# Autodesk Inventor assembly: Structure
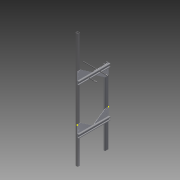
[picture p0: Inventor's stored thumbnail of the model, 180x180]
Saved by Autodesk Inventor 2015 SP1 (Build 190203100, 203)
## iProperties
Created: 2015-01-24
Part Number: Structure
Document SubType Name: Assembly
Designer: Peter
Author: Peter
## Documents named in this file (9)
- C:\Users\Brian\Documents\GitHub\FIRST-Team-1719-CAD-Team\2015 Robot CAD\Devices\Extender\Structure\Structure.iam
- C:\Users\Brian\Documents\GitHub\FIRST-Team-1719-CAD-Team\2015 Robot CAD\Lifter Super Structure\Tower\H-Shaped-Assembly\Horizontal-Unistrut-Tower-Connector-19-25.ipt
- C:\Users\Brian\Documents\GitHub\FIRST-Team-1719-CAD-Team\2015 Robot CAD\Devices\Extender\Structure\Horizontal-Unistrut-Tower-Connector-15.ipt
- C:\Users\Brian\Documents\GitHub\FIRST-Team-1719-CAD-Team\2015 Robot CAD\Devices\Extender\Structure\Square.ipt
- C:\Users\Brian\Documents\GitHub\FIRST-Team-1719-CAD-Team\2015 Robot CAD\Devices\Extender\Structure\Corner-Tower-Brace.ipt
- C:\Users\Brian\Documents\GitHub\FIRST-Team-1719-CAD-Team\2015 Robot CAD\Devices\Extender\Structure\Corner-Tower-Brace-Upper.ipt
- C:\Users\Brian\Documents\GitHub\FIRST-Team-1719-CAD-Team\2015 Robot CAD\Devices\Extender\Structure\3 8 Threaded Shaft.ipt
- C:\Users\Brian\Documents\GitHub\FIRST-Team-1719-CAD-Team\2015 Robot CAD\Devices\Extender\Structure\3 8 Threaded Shaft Pivot.ipt
- C:\Users\Brian\Documents\GitHub\FIRST-Team-1719-CAD-Team\2015 Robot CAD\Devices\Extender\Structure\3 8 Nut.ipt
## Components (18 placed, 8 different names)
1. Horizontal-Unistrut-Tower-Connector-19-25:1 — Flush:17, Mate:66, Mate:95
2. Horizontal-Unistrut-Tower-Connector-15:1 — Flush:17, Flush:18, Flush:19, Mate:73, Mate:90, Mate:92
3. Square:1 — Flush:24
4. Horizontal-Unistrut-Tower-Connector-15:2 — Flush:18, Flush:19, Mate:61, Mate:64
5. Corner-Tower-Brace:1 — Mate:61, Mate:66
6. Corner-Tower-Brace:4 — Mate:64
7. Corner-Tower-Brace-Upper:1 — Mate:73, Mate:76, Mate:86
8. Corner-Tower-Brace-Upper:2 — Mate:95, Mate:96, Mate:97
9. 3 8 Threaded Shaft:2 — Mate:76, Mate:84, Flush:25
10. 3 8 Threaded Shaft Pivot:1 — Mate:83, Flush:26, Mate:97
11. 3 8 Nut:1 — Mate:82, Mate:92
12. 3 8 Nut:2 — Mate:81, Mate:82, Mate:83, Mate:96
13. 3 8 Nut:3 — Mate:80, Flush:26
14. 3 8 Nut:4 — Mate:80, Mate:81
15. 3 8 Nut:5 — Mate:77, Mate:90
16. 3 8 Nut:6 — Mate:77, Mate:78
17. 3 8 Nut:7 — Mate:78, Mate:79, Mate:84, Mate:86
18. 3 8 Nut:8 — Mate:79, Flush:25
## Relationships (30: Mate 24, Flush 6)
- Mate:39
- Mate:40
- Mate:41
- Mate:42
- Mate:47
- Flush:17: Horizontal-Unistrut-Tower-Connector-19-25:1 ↔ Horizontal-Unistrut-Tower-Connector-15:1
- Flush:18: Horizontal-Unistrut-Tower-Connector-15:1 ↔ Horizontal-Unistrut-Tower-Connector-15:2
- Flush:19: Horizontal-Unistrut-Tower-Connector-15:1 ↔ Horizontal-Unistrut-Tower-Connector-15:2
- Mate:61: Horizontal-Unistrut-Tower-Connector-15:2 ↔ Corner-Tower-Brace:1
- Mate:64: Horizontal-Unistrut-Tower-Connector-15:2 ↔ Corner-Tower-Brace:4
- Mate:66: Horizontal-Unistrut-Tower-Connector-19-25:1 ↔ Corner-Tower-Brace:1
- Flush:24 (-12.7 mm): Square:1
- Mate:73: Horizontal-Unistrut-Tower-Connector-15:1 ↔ Corner-Tower-Brace-Upper:1
- Mate:76: Corner-Tower-Brace-Upper:1 ↔ 3 8 Threaded Shaft:2
- Mate:77: 3 8 Nut:5 ↔ 3 8 Nut:6
- Mate:78: 3 8 Nut:6 ↔ 3 8 Nut:7
- Mate:79: 3 8 Nut:7 ↔ 3 8 Nut:8
- Mate:80: 3 8 Nut:3 ↔ 3 8 Nut:4
- Mate:81: 3 8 Nut:2 ↔ 3 8 Nut:4
- Mate:82: 3 8 Nut:1 ↔ 3 8 Nut:2
- Mate:83: 3 8 Threaded Shaft Pivot:1 ↔ 3 8 Nut:2
- Mate:84: 3 8 Threaded Shaft:2 ↔ 3 8 Nut:7
- Mate:86: Corner-Tower-Brace-Upper:1 ↔ 3 8 Nut:7
- Mate:90: Horizontal-Unistrut-Tower-Connector-15:1 ↔ 3 8 Nut:5
- Mate:92: Horizontal-Unistrut-Tower-Connector-15:1 ↔ 3 8 Nut:1
- Flush:25: 3 8 Threaded Shaft:2 ↔ 3 8 Nut:8
- Flush:26: 3 8 Threaded Shaft Pivot:1 ↔ 3 8 Nut:3
- Mate:95: Horizontal-Unistrut-Tower-Connector-19-25:1 ↔ Corner-Tower-Brace-Upper:2
- Mate:96: Corner-Tower-Brace-Upper:2 ↔ 3 8 Nut:2
- Mate:97: Corner-Tower-Brace-Upper:2 ↔ 3 8 Threaded Shaft Pivot:1
